# Autodesk Inventor assembly: Baugruppe3
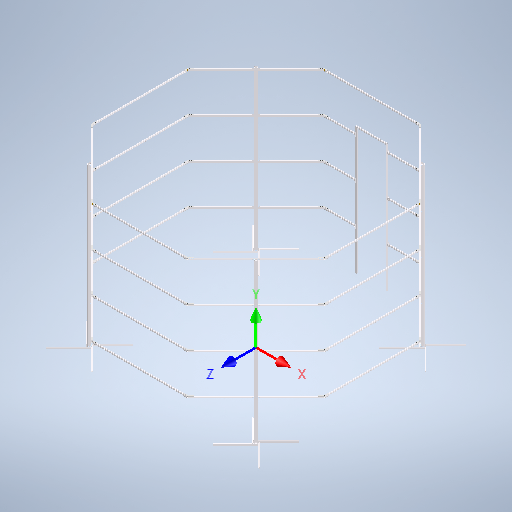
[picture p0: Inventor's stored thumbnail of the model, 512x512]
Saved by Autodesk Inventor 2025.1 (Build 291241000, 241)
## iProperties
Created: 2024-10-17
Part Number: Baugruppe3
Document SubType Name: Assembly
Designer: Kai Altwicker
Author: Kai Altwicker
## Documents named in this file (6)
- C:\Users\tallA\Repos\VolumanXR\hardware-capture\cad\rig_v2\Rig_v2.iam
- C:\Users\tallA\Repos\VolumanXR\hardware-capture\cad\rig_v1\Segment_Staender_v1.iam
- C:\Users\tallA\Repos\VolumanXR\hardware-capture\cad\rig_v1\Segment_Traeger_v1.iam
- C:\Users\tallA\Repos\VolumanXR\hardware-capture\cad\rig_v2\Verbinder_45deg_Satz.iam
- C:\Users\tallA\Repos\VolumanXR\hardware-capture\cad\rig_v1\Segment_Traeger_Tuer_v1.iam
- C:\Users\tallA\Repos\VolumanXR\hardware-capture\cad\dimensions.xlsx
## Components (72 placed, 4 different names)
1. Segment_Traeger_Tuer_v1:1 [sub-assembly] — Fluchtend:7, Fluchtend:8, Passend:7
2. Segment_Staender_v1:1 [sub-assembly] — Passend:1, Winkel:1, Passend:2, Passend:3, Fluchtend:1, Fluchtend:3, Fluchtend:5
3. Segment_Staender_v1:2 [sub-assembly] — Fluchtend:7
4. Segment_Staender_v1:3 [sub-assembly]
5. Segment_Staender_v1:4 [sub-assembly]
6. Segment_Traeger_v1:1 [sub-assembly] — Fluchtend:1, Passend:4, Fluchtend:2, Passend:5, Fluchtend:4, Passend:6, Fluchtend:6
7. Segment_Traeger_v1:2 [sub-assembly]
8. Segment_Traeger_v1:3 [sub-assembly]
9. Verbinder_45deg_Satz:2 [sub-assembly] — Passend:5, Fluchtend:3, Fluchtend:4
10. Verbinder_45deg_Satz:1 [sub-assembly] — Passend:6, Fluchtend:5, Fluchtend:6
11. Verbinder_45deg_Satz:3 [sub-assembly]
12. Verbinder_45deg_Satz:4 [sub-assembly]
13. Verbinder_45deg_Satz:5 [sub-assembly]
14. Verbinder_45deg_Satz:6 [sub-assembly]
15. Verbinder_45deg_Satz:7 [sub-assembly]
16. Verbinder_45deg_Satz:8 [sub-assembly]
17. Verbinder_45deg_Satz:9 [sub-assembly]
18. Verbinder_45deg_Satz:10 [sub-assembly]
19. Verbinder_45deg_Satz:11 [sub-assembly]
20. Verbinder_45deg_Satz:12 [sub-assembly]
21. Verbinder_45deg_Satz:13 [sub-assembly]
22. Verbinder_45deg_Satz:14 [sub-assembly]
23. Verbinder_45deg_Satz:15 [sub-assembly]
24. Verbinder_45deg_Satz:16 [sub-assembly]
25. Verbinder_45deg_Satz:17 [sub-assembly]
26. Verbinder_45deg_Satz:18 [sub-assembly]
27. Verbinder_45deg_Satz:19 [sub-assembly]
28. Verbinder_45deg_Satz:20 [sub-assembly]
29. Verbinder_45deg_Satz:21 [sub-assembly]
30. Verbinder_45deg_Satz:22 [sub-assembly]
31. Verbinder_45deg_Satz:23 [sub-assembly]
32. Verbinder_45deg_Satz:24 [sub-assembly]
33. Verbinder_45deg_Satz:25 [sub-assembly] — Fluchtend:8
34. Verbinder_45deg_Satz:26 [sub-assembly]
35. Verbinder_45deg_Satz:27 [sub-assembly]
36. Verbinder_45deg_Satz:28 [sub-assembly]
37. Verbinder_45deg_Satz:29 [sub-assembly]
38. Verbinder_45deg_Satz:30 [sub-assembly]
39. Verbinder_45deg_Satz:31 [sub-assembly]
40. Verbinder_45deg_Satz:32 [sub-assembly]
41. Verbinder_45deg_Satz:33 [sub-assembly]
42. Verbinder_45deg_Satz:34 [sub-assembly]
43. Verbinder_45deg_Satz:35 [sub-assembly]
44. Verbinder_45deg_Satz:36 [sub-assembly]
45. Verbinder_45deg_Satz:37 [sub-assembly]
46. Verbinder_45deg_Satz:38 [sub-assembly]
47. Verbinder_45deg_Satz:39 [sub-assembly]
48. Verbinder_45deg_Satz:40 [sub-assembly]
49. Verbinder_45deg_Satz:41 [sub-assembly]
50. Verbinder_45deg_Satz:42 [sub-assembly]
51. Verbinder_45deg_Satz:43 [sub-assembly]
52. Verbinder_45deg_Satz:44 [sub-assembly]
53. Verbinder_45deg_Satz:45 [sub-assembly]
54. Verbinder_45deg_Satz:46 [sub-assembly]
55. Verbinder_45deg_Satz:47 [sub-assembly]
56. Verbinder_45deg_Satz:48 [sub-assembly]
57. Verbinder_45deg_Satz:49 [sub-assembly]
58. Verbinder_45deg_Satz:50 [sub-assembly]
59. Verbinder_45deg_Satz:51 [sub-assembly]
60. Verbinder_45deg_Satz:52 [sub-assembly]
61. Verbinder_45deg_Satz:53 [sub-assembly]
62. Verbinder_45deg_Satz:54 [sub-assembly]
63. Verbinder_45deg_Satz:55 [sub-assembly]
64. Verbinder_45deg_Satz:56 [sub-assembly]
65. Verbinder_45deg_Satz:57 [sub-assembly]
66. Verbinder_45deg_Satz:58 [sub-assembly]
67. Verbinder_45deg_Satz:59 [sub-assembly]
68. Verbinder_45deg_Satz:60 [sub-assembly]
69. Verbinder_45deg_Satz:61 [sub-assembly]
70. Verbinder_45deg_Satz:62 [sub-assembly]
71. Verbinder_45deg_Satz:63 [sub-assembly]
72. Verbinder_45deg_Satz:64 [sub-assembly]
## Component patterns: (4 elements, first: Segment_Staender_v1:1), (3 elements, first: Segment_Traeger_v1:1), (2 elements), Komponentenanordnung 2:2 (2 elements), Komponentenanordnung 2:3 (2 elements), Komponentenanordnung 2:4 (2 elements), (4 elements, first: Verbinder_45deg_Satz:2 + Verbinder_45deg_Satz:1), Komponentenanordnung 1:2 (4 elements), Komponentenanordnung 1:3 (4 elements), Komponentenanordnung 1:4 (4 elements), Komponentenanordnung 1:5 (4 elements), Komponentenanordnung 1:6 (4 elements), Komponentenanordnung 1:7 (4 elements), Komponentenanordnung 1:8 (4 elements)
## Relationships (16: Flush 8, Mate 7, Angle 1)
- Passend:1 [Mate]: Segment_Staender_v1:1
- Winkel:1 [Angle] (135 deg): Segment_Staender_v1:1
- Passend:2 [Mate]: Segment_Staender_v1:1
- Passend:3 [Mate] (1810.6602 mm): Segment_Staender_v1:1
- Fluchtend:1 [Flush]: Segment_Staender_v1:1 ↔ Segment_Traeger_v1:1
- Passend:4 [Mate] (1810.6602 mm): Segment_Traeger_v1:1
- Fluchtend:2 [Flush]: Segment_Traeger_v1:1
- Passend:5 [Mate]: Segment_Traeger_v1:1 ↔ Verbinder_45deg_Satz:2
- Fluchtend:3 [Flush]: Segment_Staender_v1:1 ↔ Verbinder_45deg_Satz:2
- Fluchtend:4 [Flush]: Segment_Traeger_v1:1 ↔ Verbinder_45deg_Satz:2
- Passend:6 [Mate]: Segment_Traeger_v1:1 ↔ Verbinder_45deg_Satz:1
- Fluchtend:5 [Flush]: Segment_Staender_v1:1 ↔ Verbinder_45deg_Satz:1
- Fluchtend:6 [Flush]: Segment_Traeger_v1:1 ↔ Verbinder_45deg_Satz:1
- Fluchtend:7 [Flush]: Segment_Traeger_Tuer_v1:1 ↔ Segment_Staender_v1:2
- Fluchtend:8 [Flush]: Segment_Traeger_Tuer_v1:1 ↔ Verbinder_45deg_Satz:25
- Passend:7 [Mate]: Segment_Traeger_Tuer_v1:1
## Named parameters: d_tol = 0.3 mm, d_wand = 1.5 mm, l_profil_traeger = 1500 mm, l_profil_staender = 2500 mm, b_profil_40x40 = 40 mm, h_profil_40x40 = 40 mm, b_profil_20x20 = 20 mm, h_profil_20x20 = 20 mm, D_oct = 3621.32034 mm, d_traeger = 625 mm, l_profil_40x40 = 2500 mm, l_profil_20x20 = 1500 mm
